# Autodesk Inventor assembly: IM_Matchboxscope_plate_3 MB bg
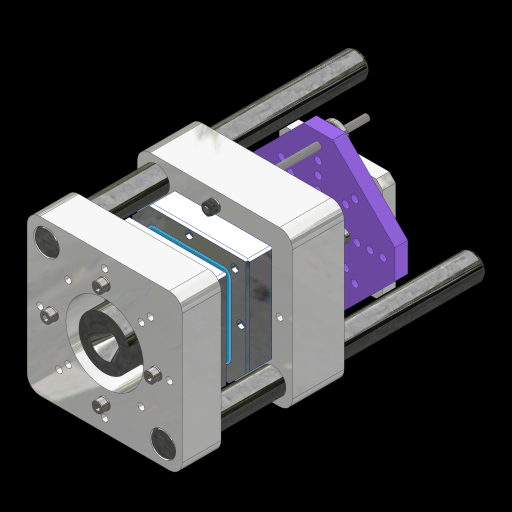
[picture p0: Inventor's stored thumbnail of the model, 512x512]
Saved by Autodesk Inventor 2024 (Build 280153000, 153)
## iProperties
Created: 2023-06-29
Part Number: IM_Matchboxscope_plate_3 MB bg
Document SubType Name: Assembly
Designer: buchmannmartin
Mass: 4335.9 g
Surface Area: 2658.93 cm^2
Volume: 1319.63 cm^3
Density: 3.28569 g/cm^3
Author: buchmannmartin
## Documents named in this file (13)
- E:\User\Dokumente\#BeneEspressoscope\IM1_Matchboxscope_plate_3 MB bg.iam
- E:\User\Dokumente\#BeneEspressoscope\MicroPlast-MB-BG.iam
- E:\User\Dokumente\#BeneEspressoscope\IM1_Matchboxscope_plate_3 MB Layout.ipt
- E:\User\Dokumente\#BeneEspressoscope\IM1_Matchboxscope_plate_3.ipt
- E:\User\Dokumente\#BeneEspressoscope\IM1-MoldTop.ipt
- E:\User\Dokumente\#BeneEspressoscope\IM1-MoldBottom.ipt
- E:\User\Dokumente\#BeneEspressoscope\Auswerfer DIN1530-AH-ISO6751-100mm.ipt
- E:\User\Dokumente\#BeneEspressoscope\D_180_13_1\D_180_13_1.ipt
- E:\User\Dokumente\Inventor\Content Center Files\R2024\de-DE\ISO 7092\ISO 7092 - ST 5 - 140 HV.ipt
- E:\User\Dokumente\Inventor\Content Center Files\R2024\de-DE\ISO 4762(2)\ISO 4762 - M5 x 50ISO.ipt
- E:\User\Dokumente\#BeneEspressoscope\ThreadedRod-M5x125.ipt
- E:\User\Dokumente\Inventor\Content Center Files\R2024\de-DE\ISO 4034(2)\ISO 4034 - M5 - ISO.ipt
- E:\User\Dokumente\Inventor\Content Center Files\R2024\de-DE\DIN 467\DIN 467 - M5.ipt
## Components (29 placed, 12 different names)
1. MicroPlast-MB-BG:1 [sub-assembly] — Passend:1, Passend:2, Passend:3, Passend:73, Passend:74, Passend:75, Passend:78, Passend:79, Passend:85, Passend:86, Passend:87, Passend:88, Passend:89, Passend:90, Passend:91, Passend:92, Passend:93, Passend:94, Fluchtend:8, Passend:98, Passend:100, Einfügen:5, Einfügen:6, Passend:108, Passend:110
2. IM1_Matchboxscope_plate_3:1 — Fluchtend:2, Fluchtend:3, Passend:65, Passend:66, Passend:80
3. IM1-MoldTop:1 — Fluchtend:2, Fluchtend:3, Fluchtend:4, Fluchtend:5, Passend:64, Passend:66, Passend:74, Passend:75, Passend:76, Passend:77
4. IM1-MoldBottom:1 — Fluchtend:4, Fluchtend:5, Passend:3, Fluchtend:6, Passend:5, Passend:64, Passend:65
5. Auswerfer DIN1530-AH-ISO6751-100mm:2 — Passend:77, Fluchtend:7, Passend:79, Passend:81, Passend:84
6. Auswerfer DIN1530-AH-ISO6751-100mm:3 — Passend:76, Fluchtend:7, Passend:78, Passend:80, Passend:82, Passend:83
7. D_180_13_1:1 — Passend:82, Passend:83
8. D_180_13_1:2 — Passend:81, Passend:84
9. ISO 7092 ST 5 - 140 HV:1 — Passend:85, Passend:86, Einfügen:1
10. ISO 4762 M5 x 50:1 — Einfügen:1
11. ISO 7092 ST 5 - 140 HV:2 — Passend:87, Passend:88, Einfügen:2
12. ISO 7092 ST 5 - 140 HV:3 — Passend:89, Passend:90, Einfügen:3
13. ISO 7092 ST 5 - 140 HV:4 — Passend:91, Passend:92, Einfügen:4
14. ISO 4762 M5 x 50:2 — Einfügen:2
15. ISO 4762 M5 x 50:3 — Einfügen:3
16. ISO 4762 M5 x 50:4 — Einfügen:4
17. ThreadedRod-M5x125:1 — Passend:94, Fluchtend:8, Fluchtend:9, Passend:95, Passend:99, Passend:104, Passend:109
18. ThreadedRod-M5x125:2 — Passend:93, Fluchtend:9, Passend:96, Passend:97, Passend:103, Passend:107
19. ISO 4034 M5:1 — Passend:95, Passend:101
20. ISO 4034 M5:2 — Passend:96, Passend:102
21. ISO 7092 ST 5 - 140 HV:5 — Passend:97, Passend:98, Passend:102
22. ISO 7092 ST 5 - 140 HV:6 — Passend:99, Passend:100, Passend:101
23. ISO 7092 ST 5 - 140 HV:7 — Einfügen:5, Passend:106
24. ISO 7092 ST 5 - 140 HV:8 — Einfügen:6, Passend:105
25. ISO 4034 M5:3 — Passend:103, Passend:106
26. ISO 4034 M5:4 — Passend:104, Passend:105
27. DIN 467 M5:1 — Passend:107, Passend:108
28. DIN 467 M5:2 — Passend:109, Passend:110
29. IM1_Matchboxscope_plate_3 MB Layout:1 — Passend:1, Fluchtend:1, Passend:2
## Relationships (60: Mate 45, Flush 9, Insert 6)
- Passend:1 [Mate]: MicroPlast-MB-BG:1 ↔ IM1_Matchboxscope_plate_3 MB Layout:1
- Fluchtend:1 [Flush]: IM1_Matchboxscope_plate_3 MB Layout:1
- Passend:2 [Mate]: MicroPlast-MB-BG:1 ↔ IM1_Matchboxscope_plate_3 MB Layout:1
- Fluchtend:2 [Flush]: IM1_Matchboxscope_plate_3:1 ↔ IM1-MoldTop:1
- Fluchtend:3 [Flush]: IM1_Matchboxscope_plate_3:1 ↔ IM1-MoldTop:1
- Fluchtend:4 [Flush]: IM1-MoldTop:1 ↔ IM1-MoldBottom:1
- Fluchtend:5 [Flush]: IM1-MoldTop:1 ↔ IM1-MoldBottom:1
- Passend:3 [Mate]: MicroPlast-MB-BG:1 ↔ IM1-MoldBottom:1
- Fluchtend:6 [Flush]: IM1-MoldBottom:1
- Passend:5 [Mate]: IM1-MoldBottom:1
- Passend:64 [Mate]: IM1-MoldTop:1 ↔ IM1-MoldBottom:1
- Passend:65 [Mate]: IM1_Matchboxscope_plate_3:1 ↔ IM1-MoldBottom:1
- Passend:66 [Mate]: IM1_Matchboxscope_plate_3:1 ↔ IM1-MoldTop:1
- Passend:73 [Mate] (-155 mm): MicroPlast-MB-BG:1
- Passend:74 [Mate]: MicroPlast-MB-BG:1 ↔ IM1-MoldTop:1
- Passend:75 [Mate] (8.2 mm): MicroPlast-MB-BG:1 ↔ IM1-MoldTop:1
- Passend:76 [Mate]: IM1-MoldTop:1 ↔ Auswerfer DIN1530-AH-ISO6751-100mm:3
- Passend:77 [Mate]: IM1-MoldTop:1 ↔ Auswerfer DIN1530-AH-ISO6751-100mm:2
- Fluchtend:7 [Flush]: Auswerfer DIN1530-AH-ISO6751-100mm:2 ↔ Auswerfer DIN1530-AH-ISO6751-100mm:3
- Passend:78 [Mate]: MicroPlast-MB-BG:1 ↔ Auswerfer DIN1530-AH-ISO6751-100mm:3
- Passend:79 [Mate] (24.8 mm): MicroPlast-MB-BG:1 ↔ Auswerfer DIN1530-AH-ISO6751-100mm:2
- Passend:80 [Mate]: IM1_Matchboxscope_plate_3:1 ↔ Auswerfer DIN1530-AH-ISO6751-100mm:3
- Passend:81 [Mate]: Auswerfer DIN1530-AH-ISO6751-100mm:2 ↔ D_180_13_1:2
- Passend:82 [Mate]: Auswerfer DIN1530-AH-ISO6751-100mm:3 ↔ D_180_13_1:1
- Passend:83 [Mate]: Auswerfer DIN1530-AH-ISO6751-100mm:3 ↔ D_180_13_1:1
- Passend:84 [Mate]: Auswerfer DIN1530-AH-ISO6751-100mm:2 ↔ D_180_13_1:2
- Passend:85 [Mate]: MicroPlast-MB-BG:1 ↔ ISO 7092 ST 5 - 140 HV:1
- Passend:86 [Mate]: MicroPlast-MB-BG:1 ↔ ISO 7092 ST 5 - 140 HV:1
- Passend:87 [Mate]: MicroPlast-MB-BG:1 ↔ ISO 7092 ST 5 - 140 HV:2
- Passend:88 [Mate]: MicroPlast-MB-BG:1 ↔ ISO 7092 ST 5 - 140 HV:2
- Passend:89 [Mate]: MicroPlast-MB-BG:1 ↔ ISO 7092 ST 5 - 140 HV:3
- Passend:90 [Mate]: MicroPlast-MB-BG:1 ↔ ISO 7092 ST 5 - 140 HV:3
- Passend:91 [Mate]: MicroPlast-MB-BG:1 ↔ ISO 7092 ST 5 - 140 HV:4
- Passend:92 [Mate]: MicroPlast-MB-BG:1 ↔ ISO 7092 ST 5 - 140 HV:4
- Einfügen:1 [Insert]: ISO 7092 ST 5 - 140 HV:1 ↔ ISO 4762 M5 x 50:1
- Einfügen:2 [Insert]: ISO 7092 ST 5 - 140 HV:2 ↔ ISO 4762 M5 x 50:2
- Einfügen:3 [Insert]: ISO 7092 ST 5 - 140 HV:3 ↔ ISO 4762 M5 x 50:3
- Einfügen:4 [Insert]: ISO 7092 ST 5 - 140 HV:4 ↔ ISO 4762 M5 x 50:4
- Passend:93 [Mate]: MicroPlast-MB-BG:1 ↔ ThreadedRod-M5x125:2
- Passend:94 [Mate]: MicroPlast-MB-BG:1 ↔ ThreadedRod-M5x125:1
- Fluchtend:8 [Flush] (-7 mm): MicroPlast-MB-BG:1 ↔ ThreadedRod-M5x125:1
- Fluchtend:9 [Flush]: ThreadedRod-M5x125:1 ↔ ThreadedRod-M5x125:2
- Passend:95 [Mate]: ThreadedRod-M5x125:1 ↔ ISO 4034 M5:1
- Passend:96 [Mate]: ThreadedRod-M5x125:2 ↔ ISO 4034 M5:2
- Passend:97 [Mate]: ThreadedRod-M5x125:2 ↔ ISO 7092 ST 5 - 140 HV:5
- Passend:98 [Mate]: MicroPlast-MB-BG:1 ↔ ISO 7092 ST 5 - 140 HV:5
- Passend:99 [Mate]: ThreadedRod-M5x125:1 ↔ ISO 7092 ST 5 - 140 HV:6
- Passend:100 [Mate]: MicroPlast-MB-BG:1 ↔ ISO 7092 ST 5 - 140 HV:6
- Passend:101 [Mate]: ISO 4034 M5:1 ↔ ISO 7092 ST 5 - 140 HV:6
- Passend:102 [Mate]: ISO 4034 M5:2 ↔ ISO 7092 ST 5 - 140 HV:5
- Einfügen:5 [Insert]: MicroPlast-MB-BG:1 ↔ ISO 7092 ST 5 - 140 HV:7
- Einfügen:6 [Insert]: MicroPlast-MB-BG:1 ↔ ISO 7092 ST 5 - 140 HV:8
- Passend:103 [Mate]: ThreadedRod-M5x125:2 ↔ ISO 4034 M5:3
- Passend:104 [Mate]: ThreadedRod-M5x125:1 ↔ ISO 4034 M5:4
- Passend:105 [Mate]: ISO 7092 ST 5 - 140 HV:8 ↔ ISO 4034 M5:4
- Passend:106 [Mate]: ISO 7092 ST 5 - 140 HV:7 ↔ ISO 4034 M5:3
- Passend:107 [Mate]: ThreadedRod-M5x125:2 ↔ DIN 467 M5:1
- Passend:108 [Mate]: MicroPlast-MB-BG:1 ↔ DIN 467 M5:1
- Passend:109 [Mate]: ThreadedRod-M5x125:1 ↔ DIN 467 M5:2
- Passend:110 [Mate]: MicroPlast-MB-BG:1 ↔ DIN 467 M5:2
